# Autodesk Inventor assembly: esp32-oled-box
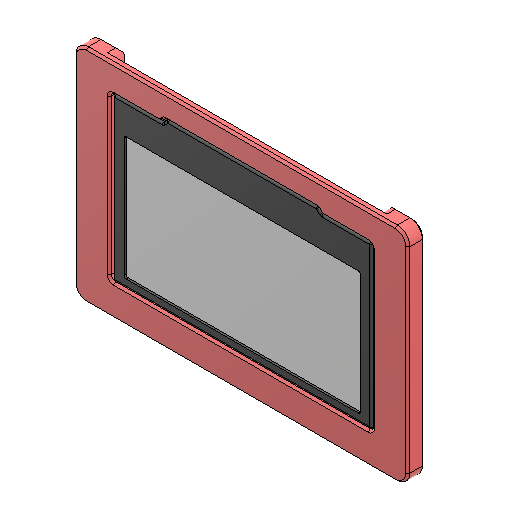
[picture p0: Inventor's stored thumbnail of the model, 512x512]
Saved by Autodesk Inventor 2026 (Build 300175050, 175E)
## iProperties
Created: 2025-06-21
Part Number: esp32-oled-box
Document SubType Name: Assembly
Designer: queezz
Author: queezz
## Documents named in this file (3)
- C:\Users\queezz\Dropbox\Drawings\PIHTI\ElectronicsBox\esp32-ambient-logger\esp32-oled-box.iam
- C:\Users\queezz\Dropbox\Drawings\PIHTI\ElectronicsBox\esp32-ambient-logger\oled-2.42-variant.iam
- C:\Users\queezz\Dropbox\Drawings\PIHTI\ElectronicsBox\esp32-ambient-logger\screen-frame.ipt
## Components (2 placed, 2 different names)
1. oled-2.42-variant:1 [sub-assembly] — Mate:2, Mate:3
2. screen-frame:1 — Mate:2, Flush:2, Mate:3
## Relationships (3: Mate 2, Flush 1)
- Mate:2: oled-2.42-variant:1 ↔ screen-frame:1
- Flush:2: screen-frame:1
- Mate:3: oled-2.42-variant:1 ↔ screen-frame:1
